# Autodesk Inventor assembly: Movable Motor
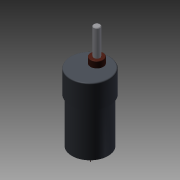
[picture p0: Inventor's stored thumbnail of the model, 180x180]
Saved by Autodesk Inventor 2015 (Build 190159000, 159)
## iProperties
Created: 2015-09-28
Part Number: Movable Motor
Document SubType Name: Assembly
Designer: Jing-Chen
Author: Jing-Chen
## Documents named in this file (3)
- C:\Users\Jing-Chen\Desktop\Bionic Hybrids 2016\Bionic-Hybrids\CAD\Drivetrain\Modified Parts\Movable Motor.iam
- C:\Users\Jing-Chen\Desktop\Bionic Hybrids 2016\Bionic-Hybrids\KOP\Tetrix_Kit_FTC\Imported Components\tetrix_739083_2012\TETRIX_739083_MOTOR_2012.ipt
- C:\Users\Jing-Chen\Desktop\Bionic Hybrids 2016\Bionic-Hybrids\KOP\Tetrix_Kit_FTC\Imported Components\tetrix_739083_2012\TETRIX_739083_AXLE_2012.ipt
## Components (2 placed, 2 different names)
1. TETRIX_739083_MOTOR_2012:1 — Mate:1, Mate:2
2. TETRIX_739083_AXLE_2012:1 — Mate:1, Mate:2
## Relationships (2: Mate 2)
- Mate:1: TETRIX_739083_MOTOR_2012:1 ↔ TETRIX_739083_AXLE_2012:1
- Mate:2: TETRIX_739083_MOTOR_2012:1 ↔ TETRIX_739083_AXLE_2012:1
